# Autodesk Inventor assembly: MIR_HbBatteryCase
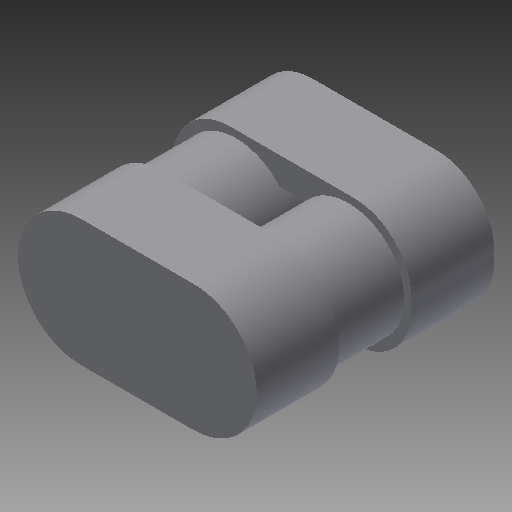
[picture p0: Inventor's stored thumbnail of the model, 512x512]
Saved by Autodesk Inventor 2018.1 (Build 221171000, 171)
## iProperties
Created: 2017-09-02
Part Number: MIR_HbBatteryCase
Material: 一般
Document SubType Name: Assembly
Designer: sktom
Author: sktom
## Documents named in this file (4)
- D:\CloudStrage\OneDrive\CAD\MAJ\hackberry\HACKberry-hardware\3D_69%inlength\Inventor\HbBatteryCase\MIR_HbBatteryCase.iam
- D:\CloudStrage\OneDrive\CAD\MAJ\hackberry\HACKberry-hardware\3D_69%inlength\Inventor\HbBatteryCase\MIR_CaseBottom_CR123A.ipt
- D:\CloudStrage\OneDrive\CAD\MAJ\hackberry\HACKberry-hardware\3D_69%inlength\Inventor\HbBatteryCase\MIR_CR2.ipt
- D:\CloudStrage\OneDrive\CAD\MAJ\hackberry\HACKberry-hardware\3D_69%inlength\Inventor\HbBatteryCase\MIR_CaseTop_CR123A.ipt
## Components (4 placed, 3 different names)
1. MIR_CaseBottom_CR123A:1 — 挿入:2, 挿入:1
2. MIR_CR2:1 — 挿入:4, 挿入:2
3. MIR_CR2:2 — 挿入:3, 挿入:1
4. MIR_CaseTop_CR123A:1 — 挿入:4, 挿入:3
## Relationships (4: Insert 4)
- 挿入:4 [Insert]: MIR_CR2:1 ↔ MIR_CaseTop_CR123A:1
- 挿入:2 [Insert]: MIR_CaseBottom_CR123A:1 ↔ MIR_CR2:1
- 挿入:3 [Insert]: MIR_CR2:2 ↔ MIR_CaseTop_CR123A:1
- 挿入:1 [Insert]: MIR_CaseBottom_CR123A:1 ↔ MIR_CR2:2
